# Autodesk Inventor assembly: SystemAssemV2
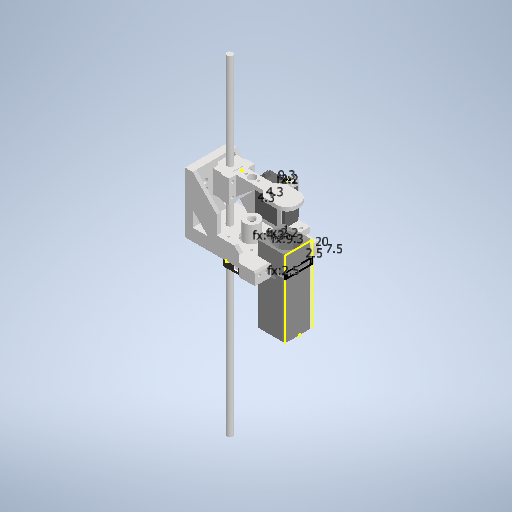
[picture p0: Inventor's stored thumbnail of the model, 512x512]
Saved by Autodesk Inventor 2025.1 (Build 291241000, 241)
## iProperties
Created: 2025-03-02
Part Number: SystemAssemV2
Document SubType Name: Assembly
Designer: 13156
Author: 13156
## Documents named in this file (10)
- C:\Users\13156\OneDrive - Binghamton University\Documents\GitHub\Perovskite-Automated-Synthesis-System\CAD\Pipette\SystemAssemV2.iam
- C:\Users\13156\OneDrive - Binghamton University\Documents\GitHub\Perovskite-Automated-Synthesis-System\CAD\Pipette\HolderV2.ipt
- C:\Users\13156\OneDrive - Binghamton University\Documents\GitHub\Perovskite-Automated-Synthesis-System\CAD\Non 3D Printed Parts\Motors and Servos\NEMA17 Stepper Motor - 26 mm.ipt
- C:\Users\13156\OneDrive - Binghamton University\Documents\GitHub\Perovskite-Automated-Synthesis-System\CAD\Pipette\Pipette Sleeve.ipt
- C:\Users\13156\OneDrive - Binghamton University\Documents\GitHub\Perovskite-Automated-Synthesis-System\CAD\Pipette\LeadScrewBase.ipt
- C:\Users\13156\OneDrive - Binghamton University\Documents\GitHub\Perovskite-Automated-Synthesis-System\CAD\Non 3D Printed Parts\Linear Rails\8mm Linear Rod.ipt
- C:\Users\13156\OneDrive - Binghamton University\Documents\GitHub\Perovskite-Automated-Synthesis-System\CAD\Non 3D Printed Parts\Linear Rails\Linear Bearing 8mm Square.ipt
- C:\Users\13156\OneDrive - Binghamton University\Documents\GitHub\Perovskite-Automated-Synthesis-System\CAD\Pipette\ActuatorV2.ipt
- C:\Users\13156\OneDrive - Binghamton University\Documents\GitHub\Perovskite-Automated-Synthesis-System\CAD\Pipette\BIGServoHolder.ipt
- C:\Users\13156\OneDrive - Binghamton University\Documents\GitHub\Perovskite-Automated-Synthesis-System\CAD\Pipette\996R.ipt
## Components (9 placed, 9 different names)
1. HolderV2:1 — Mate:1, Mate:2, Mate:3, Mate:4, Mate:5, Mate:6, Mate:7, Mate:8, Mate:9, Mate:10, Mate:13, Mate:19, Mate:20, Mate:21, Mate:26, Mate:27
2. NEMA17 Stepper Motor - 26 mm:1 — Mate:4, Mate:5, Mate:6, Mate:7, Mate:11, Mate:12
3. Pipette Sleeve:1 — Mate:8, Mate:9, Mate:10
4. LeadScrewBase:1 — Mate:11, Mate:12, Mate:18
5. 8mm Linear Rod:1 — Mate:13, Mate:14
6. Linear Bearing 8mm Square:1 — Mate:14, Mate:15, Mate:16, Mate:17
7. ActuatorV2:1 — Mate:15, Mate:16, Mate:17, Mate:18
8. BIGServoHolder:1 — Mate:19, Mate:20, Mate:21, Mate:22, Mate:23, Mate:24, Mate:25, Mate:26, Mate:27
9. 996R:1 — Mate:22, Mate:23, Mate:24, Mate:25
## Relationships (27: Mate 27)
- Mate:1: HolderV2:1
- Mate:2: HolderV2:1
- Mate:3: HolderV2:1
- Mate:4: HolderV2:1 ↔ NEMA17 Stepper Motor - 26 mm:1
- Mate:5: HolderV2:1 ↔ NEMA17 Stepper Motor - 26 mm:1
- Mate:6: HolderV2:1 ↔ NEMA17 Stepper Motor - 26 mm:1
- Mate:7: HolderV2:1 ↔ NEMA17 Stepper Motor - 26 mm:1
- Mate:8: HolderV2:1 ↔ Pipette Sleeve:1
- Mate:9: HolderV2:1 ↔ Pipette Sleeve:1
- Mate:10: HolderV2:1 ↔ Pipette Sleeve:1
- Mate:11: NEMA17 Stepper Motor - 26 mm:1 ↔ LeadScrewBase:1
- Mate:12: NEMA17 Stepper Motor - 26 mm:1 ↔ LeadScrewBase:1
- Mate:13: HolderV2:1 ↔ 8mm Linear Rod:1
- Mate:14: 8mm Linear Rod:1 ↔ Linear Bearing 8mm Square:1
- Mate:15: Linear Bearing 8mm Square:1 ↔ ActuatorV2:1
- Mate:16: Linear Bearing 8mm Square:1 ↔ ActuatorV2:1
- Mate:17: Linear Bearing 8mm Square:1 ↔ ActuatorV2:1
- Mate:18: LeadScrewBase:1 ↔ ActuatorV2:1
- Mate:19: HolderV2:1 ↔ BIGServoHolder:1
- Mate:20: HolderV2:1 ↔ BIGServoHolder:1
- Mate:21: HolderV2:1 ↔ BIGServoHolder:1
- Mate:22: BIGServoHolder:1 ↔ 996R:1
- Mate:23: BIGServoHolder:1 ↔ 996R:1
- Mate:24: BIGServoHolder:1 ↔ 996R:1
- Mate:25: BIGServoHolder:1 ↔ 996R:1
- Mate:26: HolderV2:1 ↔ BIGServoHolder:1
- Mate:27: HolderV2:1 ↔ BIGServoHolder:1
